# Autodesk Inventor assembly: handle-base
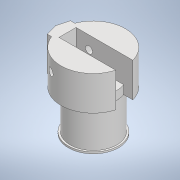
[picture p0: Inventor's stored thumbnail of the model, 180x180]
Saved by Autodesk Inventor 2021 (Build 250183000, 183)
## iProperties
Created: 2021-06-09
Part Number: handle-base
Document SubType Name: Assembly
Designer: teh18
Author: teh18
## Documents named in this file (4)
- C:\Users\teh18\OneDrive\BVE Controller\r68-bve-mascon\handle-base\handle-base.iam
- C:\Users\teh18\OneDrive\BVE Controller\r68-bve-mascon\handle-base\top.ipt
- C:\Users\teh18\OneDrive\BVE Controller\r68-bve-mascon\handle-base\bottom.ipt
- C:\Users\teh18\OneDrive\BVE Controller\r68-bve-mascon\handle_base_rod.ipt
## Components (3 placed, 3 different names)
1. top:1 — Mate:1, Mate:2, Flush:1
2. bottom:1 — Mate:1, Mate:2
3. handle_base_rod:1 — Flush:1
## Relationships (3: Mate 2, Flush 1)
- Mate:1: top:1 ↔ bottom:1
- Mate:2 (0.25 mm): top:1 ↔ bottom:1
- Flush:1: top:1 ↔ handle_base_rod:1
